# Autodesk Inventor assembly: Assembly7
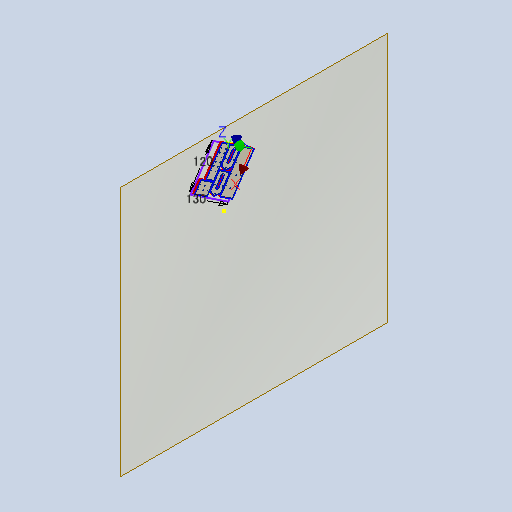
[picture p0: Inventor's stored thumbnail of the model, 512x512]
Saved by Autodesk Inventor 2025.2 (Build 292293000, 293)
## iProperties
Created: 2024-12-26
Part Number: Assembly7
Document SubType Name: Assembly
Designer: haruy
Author: haruy
## Documents named in this file (5)
- C:\Users\haruy\Documents\ロボコン\NHK2025\cad\cnc\Assembly7.iam
- C:\Users\haruy\Documents\ロボコン\NHK2025\cad\nagahisa\belt_liner\belt_liner_v1_Plate_9.ipt
- C:\Users\haruy\Documents\ロボコン\NHK2025\cad\nagahisa\belt_liner\belt_liner_v1_Plate_6.ipt
- C:\Users\haruy\Documents\ロボコン\NHK2025\cad\nagahisa\belt_liner\belt_liner_v1_Plate_2.ipt
- C:\Users\haruy\Documents\ロボコン\NHK2025\cad\nagahisa\belt_liner\belt_liner_v1_MDF_throw_plate.ipt
## Components (5 placed, 4 different names)
1. belt_liner_v1_Plate_9:1 — フラッシュ:1, メイト:3, メイト:6
2. belt_liner_v1_Plate_9:2 — フラッシュ:2, フラッシュ:7, メイト:2, フラッシュ:9, メイト:4
3. belt_liner_v1_Plate_6:1 — フラッシュ:4, メイト:5, メイト:6
4. belt_liner_v1_Plate_2:1 — フラッシュ:6, フラッシュ:7, メイト:2, メイト:3
5. belt_liner_v1_MDF_throw_plate:1 — フラッシュ:8, フラッシュ:9, メイト:4, メイト:5
## Relationships (12: Flush 7, Mate 5)
- フラッシュ:1 [Flush]: belt_liner_v1_Plate_9:1
- フラッシュ:2 [Flush]: belt_liner_v1_Plate_9:2
- フラッシュ:4 [Flush]: belt_liner_v1_Plate_6:1
- フラッシュ:6 [Flush]: belt_liner_v1_Plate_2:1
- フラッシュ:7 [Flush]: belt_liner_v1_Plate_9:2 ↔ belt_liner_v1_Plate_2:1
- メイト:2 [Mate] (5 mm): belt_liner_v1_Plate_9:2 ↔ belt_liner_v1_Plate_2:1
- フラッシュ:8 [Flush]: belt_liner_v1_MDF_throw_plate:1
- メイト:3 [Mate] (5 mm): belt_liner_v1_Plate_9:1 ↔ belt_liner_v1_Plate_2:1
- フラッシュ:9 [Flush]: belt_liner_v1_Plate_9:2 ↔ belt_liner_v1_MDF_throw_plate:1
- メイト:4 [Mate] (5 mm): belt_liner_v1_Plate_9:2 ↔ belt_liner_v1_MDF_throw_plate:1
- メイト:5 [Mate] (5 mm): belt_liner_v1_Plate_6:1 ↔ belt_liner_v1_MDF_throw_plate:1
- メイト:6 [Mate] (5 mm): belt_liner_v1_Plate_9:1 ↔ belt_liner_v1_Plate_6:1
